# Autodesk Inventor assembly: Chain Drive
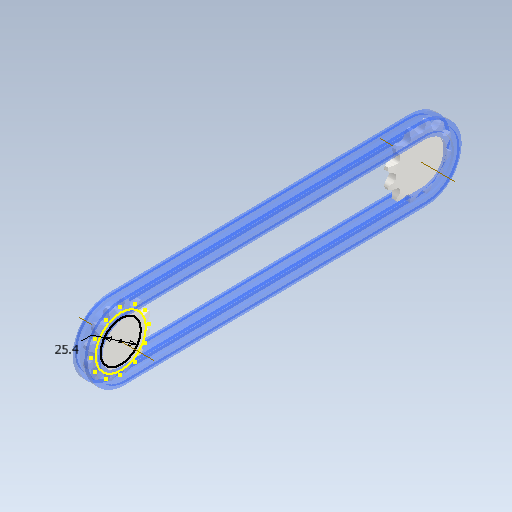
[picture p0: Inventor's stored thumbnail of the model, 512x512]
Saved by Autodesk Inventor 2020 (Build 240168000, 168)
## iProperties
ClientObjectVersion: 1
Created: 2021-01-13
Part Number: Chain Drive
Document SubType Name: Assembly
Designer: lucky
Mass: 111.065 g
Surface Area: 308.505 cm^2
Volume: 48.8702 cm^3
Density: 2.27265 g/cm^3
Author: lucky
## Documents named in this file (4)
- C:\Users\lucky\Documents\Inventor\2020DRIVEBASE\WCD_v1\Design Accelerator\Chain Drive6.iam
- C:\Users\lucky\Documents\Inventor\2020DRIVEBASE\WCD_v1\Design Accelerator\Roller Chain6.ipt
- C:\Users\lucky\Documents\Inventor\2020DRIVEBASE\WCD_v1\Design Accelerator\Roller Chain Sprocket16.ipt
- C:\Users\lucky\Documents\Inventor\2020DRIVEBASE\WCD_v1\Design Accelerator\Roller Chain Sprocket26.ipt
## Components (3 placed, 3 different names)
1. Roller Chain:1 — Flush:1, Mate:1, Mate:2, Flush:2, Mate:3, Mate:4
2. Roller Chain Sprocket1:1 — Flush:1, Mate:1, Mate:2, Rotation:1
3. Roller Chain Sprocket2:1 — Flush:2, Mate:3, Rotation:1, Mate:4
## Relationships (7: Mate 4, Flush 2, RelateRotation 1)
- Flush:1: Roller Chain:1 ↔ Roller Chain Sprocket1:1
- Mate:1: Roller Chain:1 ↔ Roller Chain Sprocket1:1
- Mate:2: Roller Chain:1 ↔ Roller Chain Sprocket1:1
- Flush:2: Roller Chain:1 ↔ Roller Chain Sprocket2:1
- Mate:3: Roller Chain:1 ↔ Roller Chain Sprocket2:1
- Rotation:1 [RelateRotation] (1 ul): Roller Chain Sprocket1:1 ↔ Roller Chain Sprocket2:1
- Mate:4: Roller Chain:1 ↔ Roller Chain Sprocket2:1
